# Autodesk Inventor assembly: Base Fall 2014
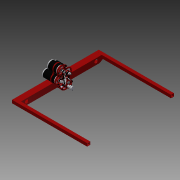
[picture p0: Inventor's stored thumbnail of the model, 180x180]
Saved by Autodesk Inventor 2013 (Build 170138000, 138)
## iProperties
Created: 2013-06-29
Part Number: Base Fall 2014
Document SubType Name: Assembly
Designer: mvarma
Author: mvarma
## Documents named in this file (10)
- C:\Users\mvarma\Desktop\GRT 2013-2014 Gearbox\Base\Base Fall 2014.iam
- C:\Users\mvarma\Desktop\GRT 2013-2014 Gearbox\Base\Box Beam\Front Support.ipt
- C:\Users\mvarma\Desktop\GRT 2013-2014 Gearbox\Base\Box Beam\Rear Support.ipt
- C:\Users\mvarma\Desktop\GRT 2013-2014 Gearbox\Base\Box Beam\Tube - Left.ipt
- C:\Users\mvarma\Desktop\GRT 2013-2014 Gearbox\Mark 4\Mark 4.5.iam
- C:\Users\mvarma\Desktop\GRT 2013-2014 Gearbox\Base\Pulleys\22T 5mm GT2 - .500 Hex Broach.ipt
- C:\Users\mvarma\Desktop\GRT 2013-2014 Gearbox\Base\Shafts\Base OutputShaft.ipt
- C:\Users\mvarma\Desktop\GRT 2013-2014 Gearbox\Base\Bearings\FR8-2RS.ipt
- C:\Users\mvarma\Desktop\GRT 2013-2014 Gearbox\Base\Bolts\Button Head Cap Screw .25-20 Thread 3.500 Length.ipt
- C:\Users\mvarma\Desktop\GRT 2013-2014 Gearbox\Base\Bolts\Large-Diameter Flat Washer .25 Screw Size.ipt
## Components (9 placed, 9 different names)
1. Tube - Left:1 — Mate:1, Mate:2, Mate:3, Mate:4, Mate:5, Mate:6, Mate:7, Mate:8, Mate:9, Mate:10, Mate:16, Mate:17
2. Front Support:1 — Mate:1, Mate:2, Mate:3
3. Rear Support:1 — Mate:4, Mate:5, Mate:6
4. Mark 4.5:1 [sub-assembly] — Mate:7, Mate:8, Mate:9, Mate:11, Mate:12, Mate:15
5. 22T 5mm GT2 - .500 Hex Broach:1 — Mate:10, Mate:11, Mate:12, Mate:13, Mate:14
6. Base OutputShaft:1 — Mate:13, Mate:14, Mate:15, Mate:20, Mate:21
7. FR8-2RS:1 — Mate:16, Mate:17
8. Button Head Cap Screw .25-20 Thread 3.500 Length:1 — Mate:18, Mate:19, Mate:20
9. Large-Diameter Flat Washer .25 Screw Size:1 — Mate:18, Mate:19, Mate:21
## Relationships (21: Mate 21)
- Mate:1: Tube - Left:1 ↔ Front Support:1
- Mate:2: Tube - Left:1 ↔ Front Support:1
- Mate:3: Tube - Left:1 ↔ Front Support:1
- Mate:4: Tube - Left:1 ↔ Rear Support:1
- Mate:5: Tube - Left:1 ↔ Rear Support:1
- Mate:6: Tube - Left:1 ↔ Rear Support:1
- Mate:7: Tube - Left:1 ↔ Mark 4.5:1
- Mate:8: Tube - Left:1 ↔ Mark 4.5:1
- Mate:9: Tube - Left:1 ↔ Mark 4.5:1
- Mate:10 (22.225 mm): Tube - Left:1 ↔ 22T 5mm GT2 - .500 Hex Broach:1
- Mate:11: Mark 4.5:1 ↔ 22T 5mm GT2 - .500 Hex Broach:1
- Mate:12: Mark 4.5:1 ↔ 22T 5mm GT2 - .500 Hex Broach:1
- Mate:13: 22T 5mm GT2 - .500 Hex Broach:1 ↔ Base OutputShaft:1
- Mate:14: 22T 5mm GT2 - .500 Hex Broach:1 ↔ Base OutputShaft:1
- Mate:15: Mark 4.5:1 ↔ Base OutputShaft:1
- Mate:16: Tube - Left:1 ↔ FR8-2RS:1
- Mate:17: Tube - Left:1 ↔ FR8-2RS:1
- Mate:18: Button Head Cap Screw .25-20 Thread 3.500 Length:1 ↔ Large-Diameter Flat Washer .25 Screw Size:1
- Mate:19: Button Head Cap Screw .25-20 Thread 3.500 Length:1 ↔ Large-Diameter Flat Washer .25 Screw Size:1
- Mate:20: Base OutputShaft:1 ↔ Button Head Cap Screw .25-20 Thread 3.500 Length:1
- Mate:21: Base OutputShaft:1 ↔ Large-Diameter Flat Washer .25 Screw Size:1
